# Autodesk Inventor assembly: BG002_huenin20_24
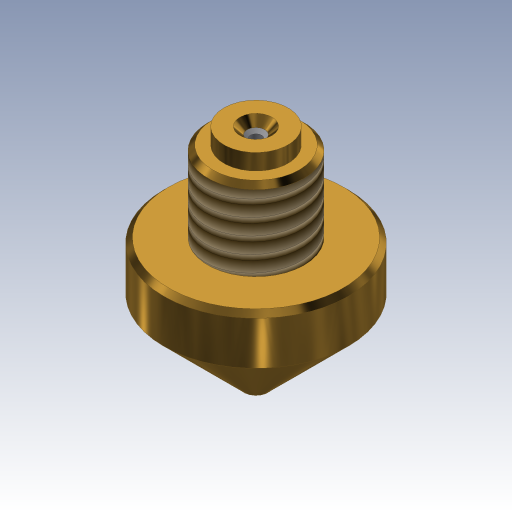
[picture p0: Inventor's stored thumbnail of the model, 512x512]
Saved by Autodesk Inventor 2023.3 (Build 273359000, 359)
## iProperties
Company: HTBLA Kaindorf
RuleStatus: InUse
Created: 2024-12-17
Part Number: BG002_huenin20_24
Project: Fiberprinter-Hotend
Material: Generisch
Description: Nozzel
Document SubType Name: Assembly
Designer: huenin20
AfterDocNew0: iProperties-Editor_aufrufen
Author: nicob
Keywords: 2024
## Documents named in this file (3)
- H:\Dokumente\Projects\Kop\Fiberprinter_Hotend\BG002_huenin20_24_Fiberprinter-Hotend_Nozzel.iam
- H:\Dokumente\Projects\Kop\Fiberprinter_Hotend\BT011_huenin20_24_Fiberprinter-Hotend_Alutube_3x0.6.ipt
- H:\Dokumente\Projects\Kop\Fiberprinter_Hotend\BT003_huenin20_23_Fiberprinter-Hotend_Nozzel_extender.ipt
## Components (2 placed, 2 different names)
1. BT011_huenin20_24_Fiberprinter-Hotend_Alutube_3x0.6:1 — Einfügen:1, Passend:1
2. BT003_huenin20_23_Fiberprinter-Hotend_Nozzel_extender:1 — Einfügen:1
## Relationships (4: Mate 2, Insert 1, Angle 1)
- Einfügen:1 [Insert]: BT011_huenin20_24_Fiberprinter-Hotend_Alutube_3x0.6:1 ↔ BT003_huenin20_23_Fiberprinter-Hotend_Nozzel_extender:1
- Passend:1 [Mate]: BT011_huenin20_24_Fiberprinter-Hotend_Alutube_3x0.6:1
- Passend:2 [Mate]
- Winkel:1 [Angle] (90 deg)
